# Autodesk Inventor assembly: Top_Backboard Assy
(part 2 of 2)
- Flush:33: Top_Backboard:1 ↔ Din97 - 4x25 - Steel Wood Screw:5
## Named parameters: d66_d33 = 0 mm, d67_d34 = 0 mm, d68_d35 = 0 mm, d69_d36 = 0 mm, d70_d33 = 0 mm, d71_d34 = 0 mm, d72_d35 = 0 mm, d73_d36 = 0 mm, d74_d33 = 0 mm, d75_d34 = 0 mm, d76_d35 = 0 mm, d77_d36 = 0 mm, d143_d133 = 8 mm, d144_d134 = 18 mm, d145_d135 = 0 mm, d146_d136 = 0 mm, d147_d137 = 0 mm, d148_d138 = 0 mm, d149_d139 = 0 mm, d150_d140 = 0 mm, d151_d141 = 0 mm, d152_d142 = 0 mm, d153_d69 = 0 mm, d154_d70 = 0 mm, d155_d71 = 0 mm, d156_d72 = 0 mm, d157_d131 = 18 mm, d158_d132 = 8 mm, d159_d133 = 8 mm, d160_d134 = 18 mm, d161_d135 = 0 mm, d162_d136 = 0 mm, d163_d137 = 0 mm, d164_d138 = 0 mm, d165_d139 = 0 mm, d166_d140 = 0 mm, d167_d141 = 0 mm, d168_d142 = 0 mm, d169_d69 = 0 mm, d170_d70 = 0 mm, d171_d71 = 0 mm, d172_d72 = 0 mm, d173_d131 = 18 mm, d174_d132 = 8 mm, d175_d133 = 8 mm, d176_d134 = 18 mm, d177_d135 = 0 mm, d178_d136 = 0 mm, d179_d137 = 0 mm, d180_d138 = 0 mm, d181_d139 = 0 mm, d182_d140 = 0 mm, d183_d141 = 0 mm, d184_d142 = 0 mm, d185_d69 = 0 mm, d186_d70 = 0 mm, d187_d71 = 0 mm, d188_d72 = 0 mm, d189_d131 = 18 mm, d190_d132 = 8 mm, d191_d133 = 8 mm, d192_d134 = 18 mm, d193_d135 = 0 mm, d194_d136 = 0 mm, d195_d137 = 0 mm, d196_d138 = 0 mm, d197_d139 = 0 mm, d198_d140 = 0 mm, d199_d141 = 0 mm, d200_d142 = 0 mm, d201_d69 = 0 mm, d202_d70 = 0 mm, d203_d71 = 0 mm, d204_d72 = 0 mm, d205_d131 = 18 mm, d206_d132 = 8 mm, d207_d133 = 8 mm, d208_d134 = 18 mm, d209_d135 = 0 mm, d210_d136 = 0 mm, d211_d137 = 0 mm, d212_d138 = 0 mm, d213_d139 = 0 mm, d214_d140 = 0 mm, d215_d141 = 0 mm, d216_d142 = 0 mm, d217_d69 = 0 mm, d218_d70 = 0 mm, d219_d71 = 0 mm, d220_d72 = 0 mm, d221_d131 = 18 mm, d222_d132 = 8 mm, d223_d133 = 8 mm, d224_d134 = 18 mm, d225_d135 = 0 mm, d226_d136 = 0 mm, d227_d137 = 0 mm, d228_d138 = 0 mm, d229_d139 = 0 mm, d230_d140 = 0 mm, d231_d141 = 0 mm, d232_d142 = 0 mm, d233_d69 = 0 mm, d234_d70 = 0 mm, d235_d71 = 0 mm, d236_d72 = 0 mm, d237_d131 = 18 mm, d238_d132 = 8 mm, d239_d133 = 8 mm, d240_d134 = 18 mm, d241_d135 = 0 mm, d242_d136 = 0 mm, d243_d137 = 0 mm, d244_d138 = 0 mm, d245_d139 = 0 mm, d246_d140 = 0 mm, d247_d141 = 0 mm, d248_d142 = 0 mm, d249_d69 = 0 mm, d250_d70 = 0 mm, d251_d71 = 0 mm, d252_d72 = 0 mm, d253_d131 = 18 mm, d254_d132 = 8 mm, d255_d133 = 8 mm, d256_d134 = 18 mm, d257_d135 = 0 mm, d258_d136 = 0 mm, d259_d137 = 0 mm, d260_d138 = 0 mm, d261_d139 = 0 mm, d262_d140 = 0 mm, d263_d141 = 0 mm, d264_d142 = 0 mm, d265_d69 = 0 mm, d266_d70 = 0 mm, d267_d71 = 0 mm, d268_d72 = 0 mm, d269_d131 = 18 mm, d270_d132 = 8 mm, d271_d133 = 8 mm, d272_d134 = 18 mm, d273_d135 = 0 mm, d274_d136 = 0 mm, d275_d137 = 0 mm, d276_d138 = 0 mm, d277_d139 = 0 mm, d278_d140 = 0 mm, d279_d141 = 0 mm, d280_d142 = 0 mm, d281_d69 = 0 mm, d282_d70 = 0 mm, d283_d71 = 0 mm, d284_d72 = 0 mm, d285_d131 = 18 mm, d286_d132 = 8 mm, d287_d133 = 8 mm, d288_d134 = 18 mm, d289_d135 = 0 mm, d290_d136 = 0 mm, d291_d137 = 0 mm, d292_d138 = 0 mm, d293_d139 = 0 mm, d294_d140 = 0 mm, d295_d141 = 0 mm, d296_d142 = 0 mm, d297_d69 = 0 mm, d298_d70 = 0 mm, d299_d71 = 0 mm, d300_d72 = 0 mm, d301_d131 = 18 mm, d302_d132 = 8 mm, d303_d133 = 8 mm, d304_d134 = 18 mm, d305_d135 = 0 mm, d306_d136 = 0 mm, d307_d137 = 0 mm, d308_d138 = 0 mm, d309_d139 = 0 mm, d310_d140 = 0 mm, d311_d141 = 0 mm, d312_d142 = 0 mm, d313_d69 = 0 mm, d314_d70 = 0 mm, d315_d71 = 0 mm, d316_d72 = 0 mm, d317_d131 = 18 mm, d318_d132 = 8 mm, d319_d133 = 8 mm, d320_d134 = 18 mm, d321_d135 = 0 mm, d322_d136 = 0 mm, d323_d137 = 0 mm, d324_d138 = 0 mm, d325_d139 = 0 mm, d326_d140 = 0 mm, d327_d141 = 0 mm, d328_d142 = 0 mm, d329_d69 = 0 mm, d330_d70 = 0 mm, d331_d71 = 0 mm, d332_d72 = 0 mm, d333_d131 = 18 mm, d334_d132 = 8 mm, d335_d133 = 8 mm, d336_d134 = 18 mm, d337_d135 = 0 mm, d338_d136 = 0 mm, d339_d137 = 0 mm, d340_d138 = 0 mm, d341_d139 = 0 mm, d342_d140 = 0 mm, d343_d141 = 0 mm, d344_d142 = 0 mm, d345_d69 = 0 mm, d346_d70 = 0 mm, d347_d71 = 0 mm, d348_d72 = 0 mm, d349_d131 = 18 mm, d350_d132 = 8 mm
